# Autodesk Inventor assembly: ESP8266-Door-Assembly
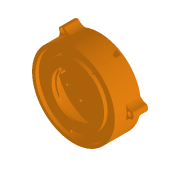
[picture p0: Inventor's stored thumbnail of the model, 180x180]
Saved by Autodesk Inventor 2020.3 (Build 243373000, 373)
## iProperties
Created: 2021-08-28
Part Number: ESP8266-Door-Assembly
Document SubType Name: Assembly
Designer: Yusuf
Mass: 154.492 g
Surface Area: 861.067 cm^2
Volume: 154.492 cm^3
Density: 1 g/cm^3
Author: Yusuf
## Documents named in this file (6)
- C:\Users\Yusuf\Desktop\BordaAcademy_BoxDesign\ESP8266-Door\ESP8266-Door-Assembly.iam
- C:\Users\Yusuf\Desktop\BordaAcademy_BoxDesign\ESP8266-Door\Door-BottomPart.ipt
- C:\Users\Yusuf\Desktop\BordaAcademy_BoxDesign\ESP8266-Door\Door-NeoPixel-24.ipt
- C:\Users\Yusuf\Desktop\BordaAcademy_BoxDesign\ESP8266-Door\Door-TopPart.ipt
- C:\Users\Yusuf\Desktop\BordaAcademy_BoxDesign\ESP8266-Door\Door-Electronics.ipt
- C:\Users\Yusuf\Desktop\BordaAcademy_BoxDesign\ESP8266-Door\Door-TopPart_MirrorV2.ipt
## Components (5 placed, 5 different names)
1. Door-BottomPart:1 — Mate:1, Mate:2, Mate:3, Mate:4, Mate:8, Mate:9, Mate:10, Mate:11, Mate:12
2. Door-NeoPixel-24:1 — Mate:6, Mate:7
3. Door-TopPart:1 — Mate:4, Mate:6, Mate:7, Mate:8
4. Door-Electronics:1 — Mate:9, Mate:13, Mate:14
5. Door-TopPart_MirrorV2:1 — Mate:10, Mate:11, Mate:12, Mate:13, Mate:14
## Relationships (13: Mate 13)
- Mate:1: Door-BottomPart:1
- Mate:2: Door-BottomPart:1
- Mate:3: Door-BottomPart:1
- Mate:4: Door-BottomPart:1 ↔ Door-TopPart:1
- Mate:6: Door-NeoPixel-24:1 ↔ Door-TopPart:1
- Mate:7: Door-NeoPixel-24:1 ↔ Door-TopPart:1
- Mate:8: Door-BottomPart:1 ↔ Door-TopPart:1
- Mate:9: Door-BottomPart:1 ↔ Door-Electronics:1
- Mate:10: Door-BottomPart:1 ↔ Door-TopPart_MirrorV2:1
- Mate:11: Door-BottomPart:1 ↔ Door-TopPart_MirrorV2:1
- Mate:12: Door-BottomPart:1 ↔ Door-TopPart_MirrorV2:1
- Mate:13: Door-Electronics:1 ↔ Door-TopPart_MirrorV2:1
- Mate:14: Door-Electronics:1 ↔ Door-TopPart_MirrorV2:1
